# Autodesk Inventor assembly: circular_dispenser
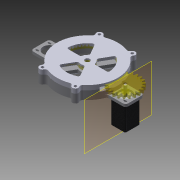
[picture p0: Inventor's stored thumbnail of the model, 180x180]
Saved by Autodesk Inventor 2014 SP2 (Build 180246200, 246)
## iProperties
Created: 2015-11-29
Part Number: circular_dispenser
Document SubType Name: Assembly
Designer: schrluka
Author: schrluka
## Documents named in this file (5)
- C:\schrluka\private\BarBot\Conception\Mechanical\Ice_Dispenser\latch_mechanics\circular_dispenser.iam
- C:\schrluka\private\BarBot\Conception\Mechanical\Ice_Dispenser\latch_mechanics\circular_funnel_top.ipt
- C:\schrluka\private\BarBot\Conception\Mechanical\Ice_Dispenser\latch_mechanics\circular_dispenser\Design Accelerator\Spur Gears2.iam
- C:\schrluka\private\BarBot\Conception\Mechanical\Ice_Dispenser\latch_mechanics\NEMA11.ipt
- C:\schrluka\private\BarBot\Conception\Mechanical\Ice_Dispenser\latch_mechanics\bottom_shield.ipt
## Components (4 placed, 4 different names)
1. circular_funnel_top:1 — Flush:1
2. Spur Gears:1 [sub-assembly] — Insert:1
3. NEMA11:1 — Insert:1
4. bottom_shield:1 — Flush:1
## Relationships (2: Insert 1, Flush 1)
- Insert:1 (20 mm): Spur Gears:1 ↔ NEMA11:1
- Flush:1: circular_funnel_top:1 ↔ bottom_shield:1
